# Autodesk Inventor assembly: Ricea f. Florentina alexandra-T7
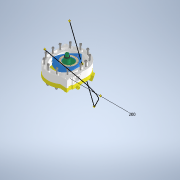
[picture p0: Inventor's stored thumbnail of the model, 180x180]
Saved by Autodesk Inventor 2022 (Build 260153000, 153)
## iProperties
Created: 2022-02-22
Part Number: Ricea f. Florentina alexandra-T7
Document SubType Name: Assembly
Designer: mtrotea
Unghi: 0,00 deg
Student_ACE: Necsulea i. M. Adrian stefanita
Grupa_ACE: CR-1.2.b
Tema_ACE: 7-Ansamblu motor Wankel
An_ACE: 2022
Author: mtrotea
## Documents named in this file (10)
- C:\Users\Alexandra\Desktop\Tema8-alexandra\Ricea f. Florentina alexandra-T7.iam
- C:\Users\Alexandra\Desktop\Tema8-alexandra\CapacSpate.ipt
- C:\Users\Alexandra\Desktop\Tema8-alexandra\StatorWankel.ipt
- C:\Users\Alexandra\Desktop\Tema8-alexandra\Arbore.ipt
- C:\Users\Alexandra\Desktop\Tema8-alexandra\SansRotor.iam
- C:\Users\Alexandra\Desktop\Tema8-alexandra\SansCapacFata.iam
- C:\Users\Alexandra\Desktop\Tema8-alexandra\Ans Suruburi Fixare.iam
- C:\Users\Alexandra\Desktop\Tema8-alexandra\Ans Pilulite Fixare.iam
- C:\Users\Alexandra\Documents\Inventor\Content Center Files\R2022\en-US\ISO 6194 1  T 1\ISO 6194_1 - Type1 22 x 35 x 7.ipt
- C:\Users\Alexandra\Desktop\Tema8-alexandra\Traseu.ipt
## Components (10 placed, 9 different names)
1. CapacSpate:1 — Mate:1, Mate:2, Angle:1, Mate:3, Mate:4, Mate:5, Mate:10
2. StatorWankel:1 — Mate:1, Mate:2, Angle:1, Animatie, Mate:7, Mate:9
3. Arbore:1 — Mate:3, Mate:4, Animatie, Mate:6, Angle:3, Rotation:1, Mate:8, Mate:11, Mate:13
4. SansRotor:1 [sub-assembly] — Mate:5, Mate:6, Angle:3, Rotation:1
5. SansCapacFata:1 [sub-assembly] — Mate:7, Mate:8, Mate:9, Mate:12
6. Ans Suruburi Fixare:1 [sub-assembly]
7. Ans Pilulite Fixare:1 [sub-assembly]
8. ISO 6194/1 Type 1 Type1 22 x 35 x 7:1 — Mate:10, Mate:11
9. ISO 6194/1 Type 1 Type1 22 x 35 x 7:2 — Mate:12, Mate:13
10. Traseu:1
## Relationships (19: Mate 13, Angle 3, Insert 2, RelateRotation 1)
- Mate:1: CapacSpate:1 ↔ StatorWankel:1
- Mate:2: CapacSpate:1 ↔ StatorWankel:1
- Angle:1 (0 deg): CapacSpate:1 ↔ StatorWankel:1
- Mate:3 (1 mm): CapacSpate:1 ↔ Arbore:1
- Mate:4: CapacSpate:1 ↔ Arbore:1
- Animatie [Angle] (0 deg): StatorWankel:1 ↔ Arbore:1
- Mate:5: CapacSpate:1 ↔ SansRotor:1
- Mate:6: Arbore:1 ↔ SansRotor:1
- Angle:3 (0 deg): Arbore:1 ↔ SansRotor:1
- Rotation:1 [RelateRotation] (3 ul): Arbore:1 ↔ SansRotor:1
- Mate:7: StatorWankel:1 ↔ SansCapacFata:1
- Mate:8: Arbore:1 ↔ SansCapacFata:1
- Mate:9: StatorWankel:1 ↔ SansCapacFata:1
- [Insert]: SansCapacFata:1 ↔ Ans Suruburi Fixare:1
- [Insert]: CapacSpate:1 ↔ Ans Pilulite Fixare:1
- Mate:10: CapacSpate:1 ↔ ISO 6194/1 Type 1 Type1 22 x 35 x 7:1
- Mate:11: Arbore:1 ↔ ISO 6194/1 Type 1 Type1 22 x 35 x 7:1
- Mate:12: SansCapacFata:1 ↔ ISO 6194/1 Type 1 Type1 22 x 35 x 7:2
- Mate:13: Arbore:1 ↔ ISO 6194/1 Type 1 Type1 22 x 35 x 7:2
